# Autodesk Inventor assembly: Palma
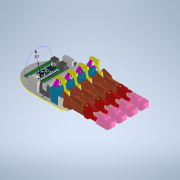
[picture p0: Inventor's stored thumbnail of the model, 180x180]
Saved by Autodesk Inventor 2020.4 (Build 244396010, 396A)
## iProperties
Created: 2021-08-20
Part Number: Palma
Document SubType Name: Assembly
Designer: chalo
Author: chalo
## Documents named in this file (10)
- C:\Users\chalo\OneDrive\Documents\GitHub\Interfaces-Biomedicas-2021\Gonzalo Palarea\Inventor\_completa\Palma.iam
- C:\Users\chalo\OneDrive\Documents\GitHub\Interfaces-Biomedicas-2021\Gonzalo Palarea\Inventor\tipo2\Prototipo2.iam
- C:\Users\chalo\OneDrive\Documents\GitHub\Interfaces-Biomedicas-2021\Gonzalo Palarea\Inventor\tipo2\Palma.ipt
- C:\Users\chalo\OneDrive\Documents\GitHub\Interfaces-Biomedicas-2021\Gonzalo Palarea\Inventor\referencias\18650.ipt
- C:\Users\chalo\OneDrive\Documents\GitHub\Interfaces-Biomedicas-2021\Gonzalo Palarea\Inventor\referencias\Battery Holder 18650_COMF_BHC-18650-1A.ipt
- C:\Users\chalo\OneDrive\Documents\GitHub\Interfaces-Biomedicas-2021\Gonzalo Palarea\Inventor\tipo2\Base_v2.ipt
- C:\Users\chalo\OneDrive\Documents\GitHub\Interfaces-Biomedicas-2021\Gonzalo Palarea\Inventor\tipo2\Metacarpo.ipt
- C:\Users\chalo\OneDrive\Documents\GitHub\Interfaces-Biomedicas-2021\Gonzalo Palarea\Inventor\tipo2\Falange_media_distal.ipt
- C:\Users\chalo\OneDrive\Documents\GitHub\Interfaces-Biomedicas-2021\Gonzalo Palarea\Inventor\servoconbrazo.iam
- C:\Users\chalo\OneDrive\Documents\GitHub\Interfaces-Biomedicas-2021\Gonzalo Palarea\Inventor\referencias\PCB_Prueba.iam
## Components (12 placed, 9 different names)
1. Prototipo2:1 [sub-assembly] — Flush:1, Flush:2, Flush:3, Mate:1, Flush:4
2. Prototipo2:2 [sub-assembly] — Flush:1, Mate:1, Mate:2, Flush:4, Flush:5, Flush:7
3. Prototipo2:3 [sub-assembly] — Flush:2, Mate:2, Mate:3, Flush:5, Flush:6
4. Prototipo2:4 [sub-assembly] — Flush:3, Mate:3, Flush:6
5. Palma:1 — Flush:7, Mate:5, Angle:1
6. 18650:2 — Mate:4, Tangent:1, Tangent:2
7. Battery Holder 18650_COMF_BHC-18650-1A:1 — Mate:4, Tangent:1, Mate:5, Tangent:2, Angle:1
8. Base_v2:1 — Insert:1, Mate:6, Insert:3
9. Metacarpo:1 — Insert:1, Insert:2
10. Falange_media_distal:1 — Insert:2
11. servoconbrazo:1 [sub-assembly] — Mate:6, Insert:3
12. PCB_Prueba:1 [sub-assembly]
## Relationships (19: Flush 7, Mate 6, Insert 3, Tangent 2, Angle 1)
- Flush:1: Prototipo2:1 ↔ Prototipo2:2
- Flush:2: Prototipo2:1 ↔ Prototipo2:3
- Flush:3: Prototipo2:1 ↔ Prototipo2:4
- Mate:1 (7 mm): Prototipo2:1 ↔ Prototipo2:2
- Mate:2 (7 mm): Prototipo2:2 ↔ Prototipo2:3
- Mate:3 (7 mm): Prototipo2:3 ↔ Prototipo2:4
- Flush:4: Prototipo2:1 ↔ Prototipo2:2
- Flush:5: Prototipo2:2 ↔ Prototipo2:3
- Flush:6: Prototipo2:3 ↔ Prototipo2:4
- Flush:7: Prototipo2:2 ↔ Palma:1
- Mate:4: 18650:2 ↔ Battery Holder 18650_COMF_BHC-18650-1A:1
- Tangent:1: 18650:2 ↔ Battery Holder 18650_COMF_BHC-18650-1A:1
- Mate:5: Palma:1 ↔ Battery Holder 18650_COMF_BHC-18650-1A:1
- Tangent:2 (1 mm): 18650:2 ↔ Battery Holder 18650_COMF_BHC-18650-1A:1
- Angle:1 (0 deg): Palma:1 ↔ Battery Holder 18650_COMF_BHC-18650-1A:1
- Insert:1: Base_v2:1 ↔ Metacarpo:1
- Insert:2: Metacarpo:1 ↔ Falange_media_distal:1
- Mate:6: Base_v2:1 ↔ servoconbrazo:1
- Insert:3: Base_v2:1 ↔ servoconbrazo:1
